# Autodesk Inventor assembly: A
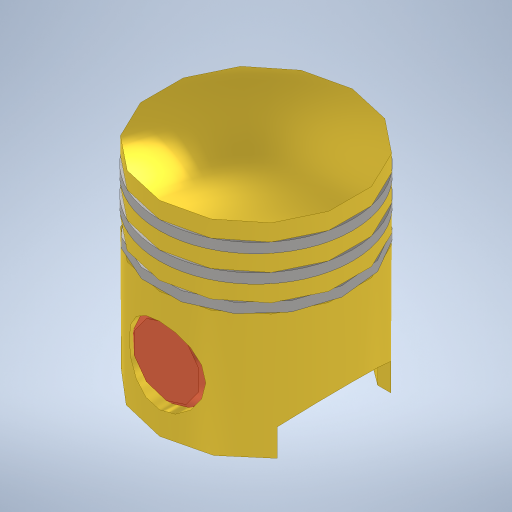
[picture p0: Inventor's stored thumbnail of the model, 512x512]
Saved by Autodesk Inventor 2023 (Build 270158000, 158)
## iProperties
Created: 2025-10-05
Part Number: A
Document SubType Name: Assembly
Designer: ayush
Author: ayush
## Documents named in this file (4)
- C:\Users\ayush\Desktop\INVENTOR FILES COLLEGE\engine\A.iam
- C:\Users\ayush\Desktop\INVENTOR FILES COLLEGE\engine\part 1 piston.ipt
- C:\Users\ayush\Desktop\INVENTOR FILES COLLEGE\engine\Part5 PISTON RING.ipt
- C:\Users\ayush\Desktop\INVENTOR FILES COLLEGE\engine\Part6 PIN.ipt
## Components (5 placed, 3 different names)
1. part 1 piston:1 — Mate:1, Mate:2, Mate:3, Mate:4, Mate:5, Mate:6, Mate:7, Tangent:1
2. Part5 PISTON RING:1 — Mate:1, Mate:6
3. Part5 PISTON RING:2 — Mate:2, Mate:5
4. Part5 PISTON RING:3 — Mate:3, Mate:4
5. Part6 PIN:1 — Mate:7, Tangent:1
## Relationships (8: Mate 7, Tangent 1)
- Mate:1: part 1 piston:1 ↔ Part5 PISTON RING:1
- Mate:2: part 1 piston:1 ↔ Part5 PISTON RING:2
- Mate:3: part 1 piston:1 ↔ Part5 PISTON RING:3
- Mate:4: part 1 piston:1 ↔ Part5 PISTON RING:3
- Mate:5: part 1 piston:1 ↔ Part5 PISTON RING:2
- Mate:6: part 1 piston:1 ↔ Part5 PISTON RING:1
- Mate:7: part 1 piston:1 ↔ Part6 PIN:1
- Tangent:1: part 1 piston:1 ↔ Part6 PIN:1
